# Autodesk Inventor assembly: Fuselage Structure Assembly
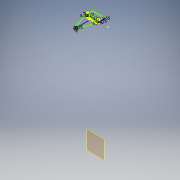
[picture p0: Inventor's stored thumbnail of the model, 180x180]
Saved by Autodesk Inventor 2018 (Build 220112000, 112)
## iProperties
Created: 2018-08-08
Part Number: Fuselage Structure Assembly
Document SubType Name: Assembly
Designer: Michael Gunderman
Author: Michael Gunderman
## Documents named in this file (5)
- C:\Users\Michael Gunderman\Documents\Special Projects\Echo 1\Echo-1-master\Echo 1\CAD work\Structures\Fuselage\Fuselage Structure Assembly.iam
- C:\Users\Michael Gunderman\Documents\Special Projects\Echo 1\Echo-1-master\Echo 1\CAD work\Preliminary Shapes\Generic Fuselage.ipt
- C:\Users\Michael Gunderman\Documents\Special Projects\Echo 1\Echo-1-master\Echo 1\CAD work\Structures\Fuselage\Fuse Structure Sketch.ipt
- C:\Users\Michael Gunderman\Documents\Special Projects\Echo 1\Echo-1-master\Echo 1\CAD work\Structures\Fuselage\Spar-Bulkhead.ipt
- C:\Users\Michael Gunderman\Documents\Special Projects\Echo 1\Echo-1-master\Echo 1\CAD work\Structures\Fuselage\Motor Mount.ipt
## Components (4 placed, 4 different names)
1. Generic Fuselage:1 — Mate:1
2. Fuse Structure Sketch:1 — Mate:3, Mate:4
3. Spar-Bulkhead:1 — Mate:2
4. Motor Mount:1 — Mate:3, Mate:4, Angle:1
## Relationships (6: Mate 4, Flush 1, Angle 1)
- Mate:1: Generic Fuselage:1
- Flush:1 (-400 mm)
- Mate:2: Spar-Bulkhead:1
- Mate:3: Fuse Structure Sketch:1 ↔ Motor Mount:1
- Mate:4: Fuse Structure Sketch:1 ↔ Motor Mount:1
- Angle:1 (180 deg): Motor Mount:1
